# Autodesk Inventor assembly: CanSat
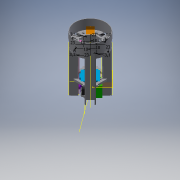
[picture p0: Inventor's stored thumbnail of the model, 180x180]
Saved by Autodesk Inventor 2018.2 (Build 222227000, 227)
## iProperties
Created: 2018-05-01
Part Number: CanSat
Document SubType Name: Assembly
Designer: suchanek
Author: suchanek
## Documents named in this file (25)
- C:\Users\Kuba\Documents\GitHub\CanSatGOSA\CanSat2.0\Schematics\Model\CanSat.iam
- C:\Users\Kuba\Documents\GitHub\CanSatGOSA\CanSat2.0\Schematics\Model\Hull_middle.ipt
- C:\Users\Kuba\Documents\GitHub\CanSatGOSA\CanSat2.0\Schematics\Model\Circuit.ipt
- C:\Users\Kuba\Documents\GitHub\CanSatGOSA\CanSat2.0\Schematics\Model\Motor_drivers.ipt
- C:\Users\Kuba\Documents\GitHub\CanSatGOSA\CanSat2.0\Schematics\Model\Hull_main.ipt
- C:\Users\Kuba\Documents\GitHub\CanSatGOSA\CanSat2.0\Schematics\Model\Circuit_center.ipt
- C:\Users\Kuba\Documents\GitHub\CanSatGOSA\CanSat2.0\Schematics\Model\Arm.ipt
- C:\Users\Kuba\Documents\GitHub\CanSatGOSA\CanSat2.0\Schematics\Model\Motor_holder.ipt
- C:\Users\Kuba\Documents\GitHub\CanSatGOSA\CanSat2.0\Schematics\Model\Motor.ipt
- C:\Users\Kuba\Documents\GitHub\CanSatGOSA\CanSat2.0\Schematics\Model\Rotor.ipt
- C:\Users\Kuba\Documents\GitHub\CanSatGOSA\CanSat2.0\Schematics\Model\Flight_controler.ipt
- C:\Users\Kuba\Documents\GitHub\CanSatGOSA\CanSat2.0\Schematics\Model\SIM808.ipt
- C:\Users\Kuba\Documents\GitHub\CanSatGOSA\CanSat2.0\Schematics\Model\Batt_pillar.ipt
- C:\Users\Kuba\Documents\GitHub\CanSatGOSA\CanSat2.0\Schematics\Model\Servo.ipt
- C:\Users\Kuba\Documents\GitHub\CanSatGOSA\CanSat2.0\Schematics\Model\Servo_bit.ipt
- C:\Users\Kuba\Documents\GitHub\CanSatGOSA\CanSat2.0\Schematics\Model\Spring.ipt
- C:\Users\Kuba\Documents\GitHub\CanSatGOSA\CanSat2.0\Schematics\Model\Scraper.ipt
- C:\Users\Kuba\Documents\GitHub\CanSatGOSA\CanSat2.0\Schematics\Model\Camera.ipt
- C:\Users\Kuba\Documents\GitHub\CanSatGOSA\CanSat2.0\Schematics\Model\Cam_SD_base.ipt
- C:\Users\Kuba\Documents\GitHub\CanSatGOSA\CanSat2.0\Schematics\Model\Cam_SD_chip.ipt
- C:\Users\Kuba\Documents\GitHub\CanSatGOSA\CanSat2.0\Schematics\Model\Hull_batt_pillar1.ipt
- C:\Users\Kuba\Documents\GitHub\CanSatGOSA\CanSat2.0\Schematics\Model\Hull_batt_pillar3.ipt
- C:\Users\Kuba\Documents\GitHub\CanSatGOSA\CanSat2.0\Schematics\Model\Hull_batt_pillar2.ipt
- C:\Users\Kuba\Documents\GitHub\CanSatGOSA\CanSat2.0\Schematics\Model\Hull_batt_pillar4.ipt
- C:\Users\Kuba\Documents\GitHub\CanSatGOSA\CanSat2.0\Schematics\Model\gamma.ipt
## Components (36 placed, 24 different names)
1. Hull_middle:1 — Rotational:2, Angle:2, Rotational:3, Flush:2, Mate:9
2. Circuit:1 — Rotational:2, Angle:2, Angle:3
3. Motor_drivers:1 — Flush:1, Angle:4, Cylindrical:1, Mate:1
4. Hull_main:1 — Rotational:3, Angle:3, Flush:1, Angle:4, Cylindrical:1, Mate:3, Mate:6, Tangent:1, Rotační:8, Rotační:9, Rotační:10, Rotační:11, Rotační:12, Rotační:13, Rotační:14, Rotační:15, Rotační:16
5. Circuit_center:1 — Flush:2, Mate:9, Tangent:1, Proti sobě:10, Proti sobě:11
6. Flight_controler:1 — Mate:1, Mate:2, Flush:4, Symmetry:1
7. SIM808:1 — Mate:2, Flush:4, Symmetry:1
8. Batt_pillar:1 — Mate:6
9. Servo:1 — Rotational:6, Flush:11, Proti sobě:16, Stejný směr:13
10. Servo_bit:1 — Rotational:6, Rigid:3, Angle:11
11. Spring:1 — Rigid:3, Rotational:7
12. Scraper:1 — Rotational:7, Angle:11
13. Camera:1 — Flush:11, Stejný směr:12, Vložit:1
14. Cam_SD_base:1 — Flush:10, Angle:13
15. Cam_SD_chip:1 — Flush:10, Angle:13
16. Hull_batt_pillar1:1 — Rotační:8, Proti sobě:18, Rotační:16
17. Hull_batt_pillar3:1 — Rotační:9, Rotační:10, Proti sobě:12, Stejný směr:12, Proti sobě:15, Vložit:1
18. Hull_batt_pillar2:1 — Rotační:11, Rotační:12
19. Hull_batt_pillar4:1 — Rotační:13, Rotační:14, Proti sobě:16, Stejný směr:13, Proti sobě:17
20. gamma:1 — Proti sobě:10, Proti sobě:11, Proti sobě:12, Proti sobě:19
21. Arm:1 — Rigid:1, Rotační:15
22. Motor_holder:1 — Rigid:1, Rigid:2
23. Motor:1 — Rigid:2, Rotational:5
24. Rotor:1 — Rotational:5
25. Arm:2
26. Motor_holder:2
27. Motor:2
28. Rotor:2
29. Arm:3
30. Motor_holder:3
31. Motor:3
32. Rotor:3
33. Arm:4
34. Motor_holder:4
35. Motor:4
36. Rotor:4
## Component patterns: (4 elements, first: Arm:1 + Motor_holder:1 + Motor:1 + Rotor:1)
## Relationships (48: Mate 15, RevoluteJoint 14, Flush 7, Angle 5, WeldJoint 3, CylindricalJoint 1, Symmetry 1, Tangent 1, Insert 1)
- Rotational:2 [RevoluteJoint]: Hull_middle:1 ↔ Circuit:1
- Angle:2 (0 deg): Hull_middle:1 ↔ Circuit:1
- Rotational:3 [RevoluteJoint]: Hull_middle:1 ↔ Hull_main:1
- Angle:3 (0 deg): Circuit:1 ↔ Hull_main:1
- Flush:1 (12 mm): Motor_drivers:1 ↔ Hull_main:1
- Angle:4 (0 deg): Motor_drivers:1 ↔ Hull_main:1
- Cylindrical:1: Motor_drivers:1 ↔ Hull_main:1
- Flush:2 (3 mm): Hull_middle:1 ↔ Circuit_center:1
- Rigid:1 [WeldJoint]: Arm:1 ↔ Motor_holder:1
- Rigid:2 [WeldJoint]: Motor_holder:1 ↔ Motor:1
- Rotational:5 [RevoluteJoint]: Motor:1 ↔ Rotor:1
- Mate:1 (5 mm): Motor_drivers:1 ↔ Flight_controler:1
- Mate:2 (2 mm): Flight_controler:1 ↔ SIM808:1
- Mate:3: Hull_main:1
- Mate:4
- Mate:5
- Flush:4 (-0.5 mm): Flight_controler:1 ↔ SIM808:1
- Mate:6: Hull_main:1 ↔ Batt_pillar:1
- Symmetry:1: Flight_controler:1 ↔ SIM808:1
- Rotational:6 [RevoluteJoint]: Servo:1 ↔ Servo_bit:1
- Rigid:3 [WeldJoint]: Servo_bit:1 ↔ Spring:1
- Rotational:7 [RevoluteJoint]: Spring:1 ↔ Scraper:1
- Angle:11 (0 deg): Servo_bit:1 ↔ Scraper:1
- Flush:10: Cam_SD_base:1 ↔ Cam_SD_chip:1
- Angle:13 (0 deg): Cam_SD_base:1 ↔ Cam_SD_chip:1
- Flush:11: Servo:1 ↔ Camera:1
- Mate:9 (0.245 mm): Hull_middle:1 ↔ Circuit_center:1
- Tangent:1 (-16.4 mm): Hull_main:1 ↔ Circuit_center:1
- Rotační:8 [RevoluteJoint]: Hull_main:1 ↔ Hull_batt_pillar1:1
- Rotační:9 [RevoluteJoint]: Hull_main:1 ↔ Hull_batt_pillar3:1
- Rotační:10 [RevoluteJoint]: Hull_main:1 ↔ Hull_batt_pillar3:1
- Rotační:11 [RevoluteJoint]: Hull_main:1 ↔ Hull_batt_pillar2:1
- Rotační:12 [RevoluteJoint]: Hull_main:1 ↔ Hull_batt_pillar2:1
- Rotační:13 [RevoluteJoint]: Hull_main:1 ↔ Hull_batt_pillar4:1
- Rotační:14 [RevoluteJoint]: Hull_main:1 ↔ Hull_batt_pillar4:1
- Proti sobě:10 [Mate] (-28 mm): Circuit_center:1 ↔ gamma:1
- Proti sobě:11 [Mate]: Circuit_center:1 ↔ gamma:1
- Proti sobě:12 [Mate] (3.163 mm): Hull_batt_pillar3:1 ↔ gamma:1
- Stejný směr:12 [Flush]: Camera:1 ↔ Hull_batt_pillar3:1
- Proti sobě:15 [Mate]: Hull_batt_pillar3:1
- Vložit:1 [Insert]: Camera:1 ↔ Hull_batt_pillar3:1
- Proti sobě:16 [Mate]: Servo:1 ↔ Hull_batt_pillar4:1
- Stejný směr:13 [Flush]: Servo:1 ↔ Hull_batt_pillar4:1
- Rotační:15 [RevoluteJoint]: Hull_main:1 ↔ Arm:1
- Proti sobě:17 [Mate]: Hull_batt_pillar4:1
- Proti sobě:18 [Mate]: Hull_batt_pillar1:1
- Proti sobě:19 [Mate]: gamma:1
- Rotační:16 [RevoluteJoint]: Hull_main:1 ↔ Hull_batt_pillar1:1
